# Autodesk Inventor assembly: Microwave Detection Region v2
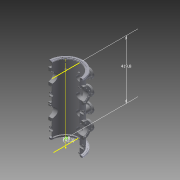
[picture p0: Inventor's stored thumbnail of the model, 180x180]
Saved by Autodesk Inventor 2015 (Build 190159000, 159)
## iProperties
Created: 2014-06-20
Part Number: Microwave Detection Region v2
Document SubType Name: Assembly
Designer: Aki
Author: Aki
## Documents named in this file (6)
- C:\ColdMatter\CADFiles\EDM Machine\Microwave Detection Region\Microwave Detection Region v2.iam
- C:\ColdMatter\CADFiles\EDM Machine\Microwave Detection Region\Detection Region Vacuum Collar v2.ipt
- C:\ColdMatter\CADFiles\EDM Machine\Microwave Detection Region\DN35CF Counter Bored.ipt
- C:\ColdMatter\CADFiles\Generic vacuum components\ISO200SS Bored K Flange.ipt
- C:\ColdMatter\CADFiles\EDM Machine\Microwave Detection Region\DN63CF Fixed Tapped Flange.ipt
- C:\ColdMatter\CADFiles\EDM Machine\Microwave Detection Region\DN16CF Fixed Tapped Flange.ipt
## Components (19 placed, 5 different names)
1. Detection Region Vacuum Collar v2:1 — Rotational:1, Rotational:2, Rotational:3, Rotational:4, Rotational:7, Rotational:8, Rotational:9, Rotational:10, Rotational:12, Mate:2, Mate:5, Mate:16, Mate:20, Mate:21, Mate:24, Mate:28, Mate:30, Mate:32, Mate:33, Mate:34, Mate:35, Mate:36, Mate:37, Mate:38, Mate:39
2. DN35CF Counter Bored:1 — Rotational:1
3. DN35CF Counter Bored:2 — Rotational:2
4. DN35CF Counter Bored:3 — Rotational:3
5. DN35CF Counter Bored:4 — Rotational:4
6. DN35CF Counter Bored:5 — Rotational:7
7. DN35CF Counter Bored:6 — Rotational:8
8. DN35CF Counter Bored:7 — Rotational:10
9. DN35CF Counter Bored:8 — Rotational:9
10. ISO200SS Bored K Flange:2 — Rotational:12
11. DN63CF Fixed Tapped Flange:1 — Mate:35, Mate:36
12. DN63CF Fixed Tapped Flange:2 — Mate:6, Mate:37
13. DN63CF Fixed Tapped Flange:3 — Mate:9, Mate:38
14. DN63CF Fixed Tapped Flange:4 — Mate:12, Mate:39
15. DN16CF Fixed Tapped Flange:1 — Mate:15, Mate:25, Mate:28
16. DN16CF Fixed Tapped Flange:2 — Mate:18, Mate:20
17. DN16CF Fixed Tapped Flange:3 — Mate:22, Mate:24
18. DN16CF Fixed Tapped Flange:4 — Mate:26, Mate:30
19. ISO200SS Bored K Flange:3 — Mate:31, Mate:33
## Relationships (43: Mate 34, RevoluteJoint 9)
- Rotational:1 [RevoluteJoint]: Detection Region Vacuum Collar v2:1 ↔ DN35CF Counter Bored:1
- Rotational:2 [RevoluteJoint]: Detection Region Vacuum Collar v2:1 ↔ DN35CF Counter Bored:2
- Rotational:3 [RevoluteJoint]: Detection Region Vacuum Collar v2:1 ↔ DN35CF Counter Bored:3
- Rotational:4 [RevoluteJoint]: Detection Region Vacuum Collar v2:1 ↔ DN35CF Counter Bored:4
- Rotational:7 [RevoluteJoint]: Detection Region Vacuum Collar v2:1 ↔ DN35CF Counter Bored:5
- Rotational:8 [RevoluteJoint]: Detection Region Vacuum Collar v2:1 ↔ DN35CF Counter Bored:6
- Rotational:9 [RevoluteJoint]: Detection Region Vacuum Collar v2:1 ↔ DN35CF Counter Bored:8
- Rotational:10 [RevoluteJoint]: Detection Region Vacuum Collar v2:1 ↔ DN35CF Counter Bored:7
- Rotational:12 [RevoluteJoint]: Detection Region Vacuum Collar v2:1 ↔ ISO200SS Bored K Flange:2
- Mate:2: Detection Region Vacuum Collar v2:1
- Mate:3
- Mate:5: Detection Region Vacuum Collar v2:1
- Mate:6: DN63CF Fixed Tapped Flange:2
- Mate:7
- Mate:9: DN63CF Fixed Tapped Flange:3
- Mate:10
- Mate:12: DN63CF Fixed Tapped Flange:4
- Mate:13
- Mate:15: DN16CF Fixed Tapped Flange:1
- Mate:16: Detection Region Vacuum Collar v2:1
- Mate:17
- Mate:18: DN16CF Fixed Tapped Flange:2
- Mate:19
- Mate:20: Detection Region Vacuum Collar v2:1 ↔ DN16CF Fixed Tapped Flange:2
- Mate:21: Detection Region Vacuum Collar v2:1
- Mate:22: DN16CF Fixed Tapped Flange:3
- Mate:23
- Mate:24: Detection Region Vacuum Collar v2:1 ↔ DN16CF Fixed Tapped Flange:3
- Mate:25: DN16CF Fixed Tapped Flange:1
- Mate:26: DN16CF Fixed Tapped Flange:4
- Mate:27
- Mate:28: Detection Region Vacuum Collar v2:1 ↔ DN16CF Fixed Tapped Flange:1
- Mate:29
- Mate:30: Detection Region Vacuum Collar v2:1 ↔ DN16CF Fixed Tapped Flange:4
- Mate:31: ISO200SS Bored K Flange:3
- Mate:32: Detection Region Vacuum Collar v2:1
- Mate:33: Detection Region Vacuum Collar v2:1 ↔ ISO200SS Bored K Flange:3
- Mate:34: Detection Region Vacuum Collar v2:1
- Mate:35: Detection Region Vacuum Collar v2:1 ↔ DN63CF Fixed Tapped Flange:1
- Mate:36: Detection Region Vacuum Collar v2:1 ↔ DN63CF Fixed Tapped Flange:1
- Mate:37: Detection Region Vacuum Collar v2:1 ↔ DN63CF Fixed Tapped Flange:2
- Mate:38: Detection Region Vacuum Collar v2:1 ↔ DN63CF Fixed Tapped Flange:3
- Mate:39: Detection Region Vacuum Collar v2:1 ↔ DN63CF Fixed Tapped Flange:4
